# Autodesk Inventor assembly: drive with fourbar linkage
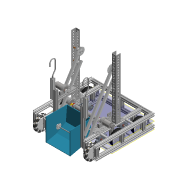
[picture p0: Inventor's stored thumbnail of the model, 180x180]
Saved by Autodesk Inventor 2013 (Build 170138000, 138)
## iProperties
Created: 2013-12-21
Part Number: drive with fourbar linkage
Document SubType Name: Assembly
Designer: kahohbein
Author: kahohbein
## Documents named in this file (27)
- C:\Users\rihoobler\Documents\GitHub\2013-2014_BlockParty\CAD\wimp with full update.iam
- C:\Users\rihoobler\Documents\GitHub\2013-2014_BlockParty\CAD\Drive\Final Drive Complete\Driveopen2.iam
- C:\Users\rihoobler\Documents\GitHub\2013-2014_BlockParty\CAD\COTSParts\Tetrix\Tetrix flat plate.ipt
- C:\Users\rihoobler\Documents\GitHub\2013-2014_BlockParty\CAD\COTSParts\Tetrix\Tetrix channel 32mm.ipt
- C:\Users\rihoobler\Documents\GitHub\2013-2014_BlockParty\CAD\COTSParts\Tetrix\Bronze bushing.ipt
- C:\Users\rihoobler\Documents\GitHub\2013-2014_BlockParty\CAD\COTSParts\Tetrix\Tetrix motor mount.ipt
- C:\Users\rihoobler\Documents\GitHub\2013-2014_BlockParty\CAD\Lift\MK3\hook prototype.ipt
- C:\Users\rihoobler\Documents\GitHub\2013-2014_BlockParty\CAD\Lift\Bosch 20x20 modified.ipt
- C:\Users\rihoobler\Documents\GitHub\2013-2014_BlockParty\CAD\four bar linkage\custom Box Aluminum.ipt
- C:\Users\rihoobler\Documents\GitHub\2013-2014_BlockParty\CAD\four bar linkage\custom bosch 8in.ipt
- C:\Users\rihoobler\Documents\GitHub\2013-2014_BlockParty\CAD\COTSParts\Tetrix\Tetrix Channel 416mm.ipt
- C:\Users\rihoobler\Documents\GitHub\2013-2014_BlockParty\CAD\COTSParts\Tetrix\Tetrix Channel 416mm_CPY.ipt
- C:\Users\rihoobler\Documents\GitHub\2013-2014_BlockParty\CAD\COTSParts\Tetrix\Tetrix Hub - axle.ipt
- C:\Users\rihoobler\Documents\GitHub\2013-2014_BlockParty\CAD\COTSParts\Tetrix\Tetrix sprocket 24T.ipt
- C:\Users\rihoobler\Documents\GitHub\2013-2014_BlockParty\CAD\Lift\MK4\Winch MK4.iam
- C:\Users\rihoobler\Documents\GitHub\2013-2014_BlockParty\CAD\COTSParts\Fasteners\4-40 SHCS x125.ipt
- C:\Users\rihoobler\Documents\GitHub\2013-2014_BlockParty\CAD\Lift\MK4\ratchet stop mk 2.ipt
- C:\Users\rihoobler\Documents\GitHub\2013-2014_BlockParty\CAD\Lift\MK4\Tetrix channel 32mm modified.ipt
- C:\Users\rihoobler\Documents\GitHub\2013-2014_BlockParty\CAD\Pick-up Blocks\axle.ipt
- C:\Users\rihoobler\Documents\GitHub\2013-2014_BlockParty\CAD\COTSParts\Tetrix\Tetrix sprocket 16T_MIR2.ipt
- C:\Users\rihoobler\Documents\GitHub\2013-2014_BlockParty\CAD\COTSParts\Tetrix\Tetrix Hub - axle_MIR2.ipt
- C:\Users\rihoobler\Documents\GitHub\2013-2014_BlockParty\CAD\COTSParts\Bosch Extrusion\Gusset 20x20 w screws.ipt
- C:\Users\rihoobler\Documents\GitHub\2013-2014_BlockParty\CAD\four bar linkage\Motor Mount Bar.ipt
- C:\Users\rihoobler\Documents\GitHub\2013-2014_BlockParty\CAD\COTSParts\Tetrix\Tetrix motor mount_MIR2.ipt
- C:\Users\rihoobler\Documents\GitHub\2013-2014_BlockParty\CAD\COTSParts\Tetrix\Tetrix motor_MIR1.ipt
- C:\Users\rihoobler\Documents\GitHub\2013-2014_BlockParty\CAD\COTSParts\Tetrix\Tetrix hub - motor.ipt
- C:\Users\rihoobler\Documents\GitHub\2013-2014_BlockParty\CAD\four bar linkage\Bucket.ipt
## Components (49 placed, 26 different names)
1. Driveopen2:1 [sub-assembly] — Mate:1, Mate:2, Mate:3, Mate:4, Mate:5, Mate:6
2. Tetrix flat plate:1 — Mate:2, Mate:3, Mate:4, Mate:15, Mate:16, Mate:110, Flush:10, Mate:184, Mate:191, Mate:192, Mate:193, Mate:201, Mate:202
3. Tetrix flat plate:2 — Mate:1, Mate:5, Mate:6, Mate:11, Mate:12, Mate:100, Flush:8, Mate:176, Mate:194, Mate:195, Mate:196, Mate:199, Mate:200
4. Tetrix channel 32mm:1 — Mate:15, Mate:16, Flush:9, Mate:111, Flush:10
5. Tetrix channel 32mm:2 — Mate:11, Mate:12, Mate:101, Flush:7, Flush:8
6. Bronze bushing:6 — Mate:102, Mate:104
7. Bronze bushing:12 — Mate:103, Mate:105
8. hook prototype:1 — Mate:80, Mate:81, Angle:1
9. Bosch 20x20 modified:1 — Mate:80, Mate:81, Mate:99, Flush:6, Flush:11, Angle:1
10. custom Box Aluminum:1 — Flush:5, Mate:96, Mate:148, Mate:151, Mate:152
11. custom Box Aluminum:3 — Flush:5, Mate:134, Mate:155, Mate:156
12. custom Box Aluminum:4 — Flush:4, Mate:124, Mate:126, Mate:129, Mate:130, Mate:131, Mate:135, Mate:207
13. custom bosch 8in:1 — Mate:96, Mate:97, Mate:99, Flush:6, Flush:11, Flush:15, Mate:206, Mate:209, Mate:210, Mate:222, Angle:3, Flush:19, Flush:20
14. Tetrix Channel 416mm:1 — Mate:100, Mate:101, Flush:7, Mate:102, Mate:103, Mate:104, Mate:105, Mate:140, Mate:141, Mate:142, Mate:148, Mate:149, Mate:150
15. Tetrix Channel 416mm_CPY:1 — Mate:110, Flush:9, Mate:111, Mate:132, Mate:133, Mate:153, Mate:154
16. Tetrix Hub - axle:1 — Mate:124, Mate:128, Mate:129, Mate:131, Mate:132, Mate:133
17. Tetrix sprocket 24T:1 — Mate:126, Mate:128, Mate:130
18. custom bosch 8in:2 — Mate:134, Mate:135, Mate:137, Flush:12, Flush:13, Mate:207, Mate:208, Mate:211, Flush:16
19. Bosch 20x20 modified:2 — Mate:137, Flush:12, Flush:13, Mate:138, Mate:139, Angle:2
20. hook prototype:2 — Mate:138, Mate:139, Angle:2
21. Tetrix Hub - axle:2 — Mate:141, Mate:142, Mate:143, Mate:144
22. Tetrix sprocket 24T:2 — Mate:145, Mate:146, Mate:147
23. Tetrix Hub - axle:3 — Mate:149, Mate:150, Mate:151, Mate:152
24. Tetrix Hub - axle:4 — Mate:153, Mate:154, Mate:155, Mate:156
25. Winch MK4:1 [sub-assembly] — Mate:197, Mate:198, Flush:14
26. 4-40 SHCS x125:1 — Mate:179, Mate:181
27. ratchet stop mk 2:1 — Mate:177, Mate:182
28. 4-40 SHCS x125:2 — Mate:178, Mate:180
29. Tetrix channel 32mm modified:1 — Mate:176, Mate:177, Mate:178, Mate:179, Mate:180, Mate:181, Mate:182, Mate:199, Mate:200
30. Tetrix channel 32mm modified:2 — Mate:184, Mate:185, Mate:186, Mate:187, Mate:188, Mate:189, Mate:190, Mate:201, Mate:202
31. ratchet stop mk 2:2 — Mate:187, Mate:188, Flush:14
32. 4-40 SHCS x125:3 — Mate:185, Mate:189
33. 4-40 SHCS x125:4 — Mate:186, Mate:190
34. Tetrix motor mount:1 — Mate:191, Mate:192, Mate:193, Mate:198
35. Tetrix motor mount:2 — Mate:194, Mate:195, Mate:196, Mate:197
36. Bronze bushing:13 — Mate:208, Mate:211, Mate:212, Mate:226
37. Bronze bushing:14 — Mate:209, Mate:210, Mate:217
38. axle:1 — Mate:212, Flush:16, Mate:216, Mate:227
39. Tetrix sprocket 16T_MIR2:1 — Mate:213, Mate:214, Mate:215
40. Tetrix Hub - axle_MIR2:1 — Mate:213, Mate:214, Mate:215, Mate:216, Mate:217
41. Gusset 20x20 w screws:1 — Mate:220, Flush:18, Mate:221
42. Gusset 20x20 w screws:2 — Mate:218, Flush:17, Mate:219, Mate:222, Mate:225
43. Motor Mount Bar:1 — Mate:218, Flush:17, Mate:219, Mate:220, Flush:18, Mate:221, Angle:3, Flush:19, Flush:20, Mate:223, Mate:224
44. Tetrix motor mount_MIR2:1 — Mate:223, Mate:224, Mate:225, Insert:1
45. Tetrix motor_MIR1:1 — Insert:1, Insert:3
46. Tetrix sprocket 16T_MIR2:2 — Insert:2
47. Tetrix hub - motor:1 — Insert:2, Insert:3
48. Bucket:1 — Mate:226, Mate:227
49. custom Box Aluminum:2 — Flush:4, Mate:97, Mate:140, Mate:143, Mate:144, Mate:145, Mate:146, Mate:147, Mate:206
## Relationships (124: Mate 101, Flush 17, Angle 3, Insert 3)
- Mate:1: Driveopen2:1 ↔ Tetrix flat plate:2
- Mate:2: Driveopen2:1 ↔ Tetrix flat plate:1
- Mate:3 (139.7 mm): Driveopen2:1 ↔ Tetrix flat plate:1
- Mate:4 (63.5 mm): Driveopen2:1 ↔ Tetrix flat plate:1
- Mate:5 (139.7 mm): Driveopen2:1 ↔ Tetrix flat plate:2
- Mate:6 (63.5 mm): Driveopen2:1 ↔ Tetrix flat plate:2
- Mate:11: Tetrix flat plate:2 ↔ Tetrix channel 32mm:2
- Mate:12: Tetrix flat plate:2 ↔ Tetrix channel 32mm:2
- Mate:15: Tetrix flat plate:1 ↔ Tetrix channel 32mm:1
- Mate:16: Tetrix flat plate:1 ↔ Tetrix channel 32mm:1
- Mate:80: hook prototype:1 ↔ Bosch 20x20 modified:1
- Mate:81: hook prototype:1 ↔ Bosch 20x20 modified:1
- Flush:4: custom Box Aluminum:4 ↔ custom Box Aluminum:2
- Flush:5: custom Box Aluminum:1 ↔ custom Box Aluminum:3
- Mate:96: custom Box Aluminum:1 ↔ custom bosch 8in:1
- Mate:97: custom bosch 8in:1 ↔ custom Box Aluminum:2
- Mate:99: Bosch 20x20 modified:1 ↔ custom bosch 8in:1
- Flush:6: Bosch 20x20 modified:1 ↔ custom bosch 8in:1
- Mate:100: Tetrix flat plate:2 ↔ Tetrix Channel 416mm:1
- Mate:101: Tetrix channel 32mm:2 ↔ Tetrix Channel 416mm:1
- Flush:7: Tetrix channel 32mm:2 ↔ Tetrix Channel 416mm:1
- Flush:8: Tetrix flat plate:2 ↔ Tetrix channel 32mm:2
- Mate:102: Bronze bushing:6 ↔ Tetrix Channel 416mm:1
- Mate:103: Bronze bushing:12 ↔ Tetrix Channel 416mm:1
- Mate:104: Bronze bushing:6 ↔ Tetrix Channel 416mm:1
- Mate:105: Bronze bushing:12 ↔ Tetrix Channel 416mm:1
- Mate:110: Tetrix flat plate:1 ↔ Tetrix Channel 416mm_CPY:1
- Flush:9: Tetrix channel 32mm:1 ↔ Tetrix Channel 416mm_CPY:1
- Mate:111: Tetrix channel 32mm:1 ↔ Tetrix Channel 416mm_CPY:1
- Flush:10: Tetrix flat plate:1 ↔ Tetrix channel 32mm:1
- Flush:11 (60.833 mm): Bosch 20x20 modified:1 ↔ custom bosch 8in:1
- Mate:124: custom Box Aluminum:4 ↔ Tetrix Hub - axle:1
- Mate:126: custom Box Aluminum:4 ↔ Tetrix sprocket 24T:1
- Mate:128: Tetrix Hub - axle:1 ↔ Tetrix sprocket 24T:1
- Mate:129: custom Box Aluminum:4 ↔ Tetrix Hub - axle:1
- Mate:130: custom Box Aluminum:4 ↔ Tetrix sprocket 24T:1
- Mate:131: custom Box Aluminum:4 ↔ Tetrix Hub - axle:1
- Mate:132: Tetrix Channel 416mm_CPY:1 ↔ Tetrix Hub - axle:1
- Mate:133: Tetrix Channel 416mm_CPY:1 ↔ Tetrix Hub - axle:1
- Mate:134: custom Box Aluminum:3 ↔ custom bosch 8in:2
- Mate:135: custom Box Aluminum:4 ↔ custom bosch 8in:2
- Mate:137: custom bosch 8in:2 ↔ Bosch 20x20 modified:2
- Flush:12: custom bosch 8in:2 ↔ Bosch 20x20 modified:2
- Flush:13 (-60.833 mm): custom bosch 8in:2 ↔ Bosch 20x20 modified:2
- Mate:138: Bosch 20x20 modified:2 ↔ hook prototype:2
- Mate:139 (-15.24 mm): Bosch 20x20 modified:2 ↔ hook prototype:2
- Mate:140: Tetrix Channel 416mm:1 ↔ custom Box Aluminum:2
- Mate:141: Tetrix Channel 416mm:1 ↔ Tetrix Hub - axle:2
- Mate:142: Tetrix Channel 416mm:1 ↔ Tetrix Hub - axle:2
- Mate:143: Tetrix Hub - axle:2 ↔ custom Box Aluminum:2
- Mate:144: Tetrix Hub - axle:2 ↔ custom Box Aluminum:2
- Mate:145: Tetrix sprocket 24T:2 ↔ custom Box Aluminum:2
- Mate:146: Tetrix sprocket 24T:2 ↔ custom Box Aluminum:2
- Mate:147: Tetrix sprocket 24T:2 ↔ custom Box Aluminum:2
- Mate:148: custom Box Aluminum:1 ↔ Tetrix Channel 416mm:1
- Mate:149: Tetrix Channel 416mm:1 ↔ Tetrix Hub - axle:3
- Mate:150: Tetrix Channel 416mm:1 ↔ Tetrix Hub - axle:3
- Mate:151: custom Box Aluminum:1 ↔ Tetrix Hub - axle:3
- Mate:152: custom Box Aluminum:1 ↔ Tetrix Hub - axle:3
- Mate:153: Tetrix Channel 416mm_CPY:1 ↔ Tetrix Hub - axle:4
- Mate:154: Tetrix Channel 416mm_CPY:1 ↔ Tetrix Hub - axle:4
- Mate:155: custom Box Aluminum:3 ↔ Tetrix Hub - axle:4
- Mate:156: custom Box Aluminum:3 ↔ Tetrix Hub - axle:4
- Mate:176: Tetrix flat plate:2 ↔ Tetrix channel 32mm modified:1
- Mate:177: ratchet stop mk 2:1 ↔ Tetrix channel 32mm modified:1
- Mate:178: 4-40 SHCS x125:2 ↔ Tetrix channel 32mm modified:1
- Mate:179: 4-40 SHCS x125:1 ↔ Tetrix channel 32mm modified:1
- Mate:180: 4-40 SHCS x125:2 ↔ Tetrix channel 32mm modified:1
- Mate:181: 4-40 SHCS x125:1 ↔ Tetrix channel 32mm modified:1
- Mate:182: ratchet stop mk 2:1 ↔ Tetrix channel 32mm modified:1
- Mate:184: Tetrix flat plate:1 ↔ Tetrix channel 32mm modified:2
- Mate:185: Tetrix channel 32mm modified:2 ↔ 4-40 SHCS x125:3
- Mate:186: Tetrix channel 32mm modified:2 ↔ 4-40 SHCS x125:4
- Mate:187: Tetrix channel 32mm modified:2 ↔ ratchet stop mk 2:2
- Mate:188: Tetrix channel 32mm modified:2 ↔ ratchet stop mk 2:2
- Mate:189: Tetrix channel 32mm modified:2 ↔ 4-40 SHCS x125:3
- Mate:190: Tetrix channel 32mm modified:2 ↔ 4-40 SHCS x125:4
- Mate:191: Tetrix flat plate:1 ↔ Tetrix motor mount:1
- Mate:192: Tetrix flat plate:1 ↔ Tetrix motor mount:1
- Mate:193: Tetrix flat plate:1 ↔ Tetrix motor mount:1
- Mate:194: Tetrix flat plate:2 ↔ Tetrix motor mount:2
- Mate:195: Tetrix flat plate:2 ↔ Tetrix motor mount:2
- Mate:196: Tetrix flat plate:2 ↔ Tetrix motor mount:2
- Mate:197: Winch MK4:1 ↔ Tetrix motor mount:2
- Mate:198: Winch MK4:1 ↔ Tetrix motor mount:1
- Mate:199: Tetrix flat plate:2 ↔ Tetrix channel 32mm modified:1
- Mate:200: Tetrix flat plate:2 ↔ Tetrix channel 32mm modified:1
- Mate:201: Tetrix flat plate:1 ↔ Tetrix channel 32mm modified:2
- Mate:202: Tetrix flat plate:1 ↔ Tetrix channel 32mm modified:2
- Flush:14: Winch MK4:1 ↔ ratchet stop mk 2:2
- Angle:1 (90 deg): hook prototype:1 ↔ Bosch 20x20 modified:1
- Angle:2 (90 deg): Bosch 20x20 modified:2 ↔ hook prototype:2
- Flush:15 (85.9981 mm): custom bosch 8in:1
- Mate:206: custom bosch 8in:1 ↔ custom Box Aluminum:2
- Mate:207: custom Box Aluminum:4 ↔ custom bosch 8in:2
- Mate:208: custom bosch 8in:2 ↔ Bronze bushing:13
- Mate:209: custom bosch 8in:1 ↔ Bronze bushing:14
- Mate:210: custom bosch 8in:1 ↔ Bronze bushing:14
- Mate:211: custom bosch 8in:2 ↔ Bronze bushing:13
- Mate:212: Bronze bushing:13 ↔ axle:1
- Flush:16 (-17.8308 mm): custom bosch 8in:2 ↔ axle:1
- Mate:213: Tetrix sprocket 16T_MIR2:1 ↔ Tetrix Hub - axle_MIR2:1
- Mate:214: Tetrix sprocket 16T_MIR2:1 ↔ Tetrix Hub - axle_MIR2:1
- Mate:215: Tetrix sprocket 16T_MIR2:1 ↔ Tetrix Hub - axle_MIR2:1
- Mate:216: axle:1 ↔ Tetrix Hub - axle_MIR2:1
- Mate:217 (3.175 mm): Bronze bushing:14 ↔ Tetrix Hub - axle_MIR2:1
- Mate:218: Gusset 20x20 w screws:2 ↔ Motor Mount Bar:1
- Flush:17: Gusset 20x20 w screws:2 ↔ Motor Mount Bar:1
- Mate:219: Gusset 20x20 w screws:2 ↔ Motor Mount Bar:1
- Mate:220: Gusset 20x20 w screws:1 ↔ Motor Mount Bar:1
- Flush:18: Gusset 20x20 w screws:1 ↔ Motor Mount Bar:1
- Mate:221: Gusset 20x20 w screws:1 ↔ Motor Mount Bar:1
- Mate:222: custom bosch 8in:1 ↔ Gusset 20x20 w screws:2
- Angle:3 (0 deg): custom bosch 8in:1 ↔ Motor Mount Bar:1
- Flush:19: custom bosch 8in:1 ↔ Motor Mount Bar:1
- Flush:20 (50.8 mm): custom bosch 8in:1 ↔ Motor Mount Bar:1
- Mate:223: Motor Mount Bar:1 ↔ Tetrix motor mount_MIR2:1
- Mate:224: Motor Mount Bar:1 ↔ Tetrix motor mount_MIR2:1
- Mate:225: Gusset 20x20 w screws:2 ↔ Tetrix motor mount_MIR2:1
- Insert:1: Tetrix motor mount_MIR2:1 ↔ Tetrix motor_MIR1:1
- Insert:2: Tetrix sprocket 16T_MIR2:2 ↔ Tetrix hub - motor:1
- Insert:3: Tetrix motor_MIR1:1 ↔ Tetrix hub - motor:1
- Mate:226: Bronze bushing:13 ↔ Bucket:1
- Mate:227: axle:1 ↔ Bucket:1
